# Autodesk Inventor assembly: UltrasonicSensor2
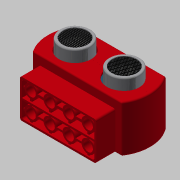
[picture p0: Inventor's stored thumbnail of the model, 180x180]
Saved by Autodesk Inventor 2019.3 (Build 233278000, 278)
## iProperties
Created: 2019-02-04
Part Number: UltrasonicSensor2
Document SubType Name: Assembly
Designer: Varga Daniel
Sending System: SolidWorks 2018
Last Author: david
Last Saved: 2019-02-07
Author: Varga Daniel
## Documents named in this file (4)
- C:\!_Dani\!_cloud\OneDrive\!_munka\Revolution\RevvyDemoKit\Structural parts\Demo parts\Ultrasonic sensor\Inventor imported\UltrasonicSensor2.iam
- C:\!_Dani\!_cloud\OneDrive\!_munka\Revolution\RevvyDemoKit\Structural parts\Demo parts\Ultrasonic sensor\Inventor imported\case.ipt
- C:\!_Dani\!_cloud\OneDrive\!_munka\Revolution\RevvyDemoKit\Structural parts\Demo parts\Ultrasonic sensor\Inventor imported\HC-SR04.ipt
- C:\!_Dani\!_cloud\OneDrive\!_munka\Revolution\RevvyDemoKit\Structural parts\Demo parts\Ultrasonic sensor\Inventor imported\rj45_vert.ipt
## Components (3 placed, 3 different names)
1. case:1 — Angle:1, Mate:1, Mate:2, Flush:1, Mate:3, Mate:4
2. HC-SR04:1 — Angle:1, Mate:1, Mate:2
3. rj45_vert:1 — Flush:1, Mate:3, Mate:4
## Relationships (6: Mate 4, Angle 1, Flush 1)
- Angle:1 (0 deg): case:1 ↔ HC-SR04:1
- Mate:1: case:1 ↔ HC-SR04:1
- Mate:2 (1 mm): case:1 ↔ HC-SR04:1
- Flush:1: case:1 ↔ rj45_vert:1
- Mate:3: case:1 ↔ rj45_vert:1
- Mate:4: case:1 ↔ rj45_vert:1
